# Autodesk Inventor assembly: USB_C_PD_PPS_sink_with_enclosure
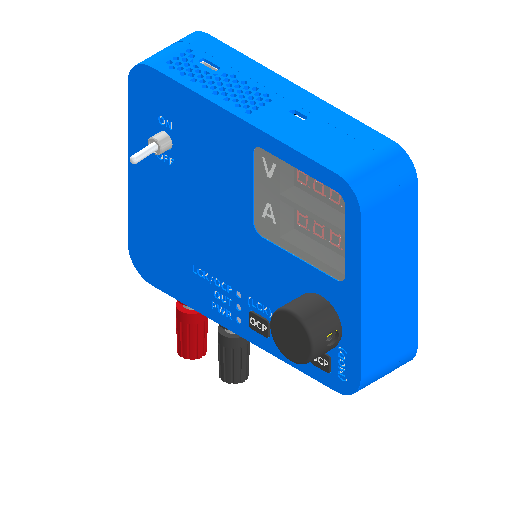
[picture p0: Inventor's stored thumbnail of the model, 512x512]
Saved by Autodesk Inventor 2025 (Build 290162000, 162)
## iProperties
Created: 2024-12-02
Part Number: USB_C_PD_PPS_sink_with_enclosure
Document SubType Name: Assembly
Designer: Jan Mareš
Author: Jan Mareš
## Documents named in this file (13)
- C:\Users\Jan Mareš\OneDrive - Vysoké učení technické v Brně\Dokumenty\Inventor\DP_PPS_USB_PD_enclosure\USB_C_PD_PPS_sink_with_enclosure.iam
- C:\Users\Jan Mareš\OneDrive - Vysoké učení technické v Brně\Dokumenty\Inventor\DP_PPS_USB_PD_enclosure\USB_C_PD_PPS_sink.iam
- C:\Users\Jan Mareš\OneDrive - Vysoké učení technické v Brně\Dokumenty\Inventor\DP_PPS_USB_PD_enclosure\top_enclosure.ipt
- C:\Users\Jan Mareš\OneDrive - Vysoké učení technické v Brně\Dokumenty\Inventor\DP_PPS_USB_PD_enclosure\STAUBLI_PK4-T_10017932.ipt
- C:\Users\Jan Mareš\OneDrive - Vysoké učení technické v Brně\Dokumenty\Inventor\DP_PPS_USB_PD_enclosure\Button cap.ipt
- C:\Users\Jan Mareš\OneDrive - Vysoké učení technické v Brně\Dokumenty\Inventor\DP_PPS_USB_PD_enclosure\Plexi-glass.ipt
- C:\Users\Jan Mareš\OneDrive - Vysoké učení technické v Brně\Dokumenty\Inventor\DP_PPS_USB_PD_enclosure\bottom_enclosure.ipt
- C:\Users\Jan Mareš\OneDrive - Vysoké učení technické v Brně\Dokumenty\Inventor\DP_PPS_USB_PD_enclosure\Aluminium_knob.ipt
- C:\Users\Jan Mareš\OneDrive - Vysoké učení technické v Brně\Dokumenty\Inventor\DP_PPS_USB_PD_enclosure\display_cover_2.ipt
- C:\Users\Jan Mareš\OneDrive - Vysoké učení technické v Brně\Dokumenty\Inventor\DP_PPS_USB_PD_enclosure\A_letter.ipt
- C:\Users\Jan Mareš\OneDrive - Vysoké učení technické v Brně\Dokumenty\Inventor\DP_PPS_USB_PD_enclosure\V_letter.ipt
- C:\Users\Jan Mareš\OneDrive - Vysoké učení technické v Brně\Dokumenty\Inventor\DP_PPS_USB_PD_enclosure\tilt_leg.ipt
- C:\Users\Jan Mareš\OneDrive - Vysoké učení technické v Brně\Dokumenty\Inventor\DP_PPS_USB_PD_enclosure\STAUBLI_PK4-T_10017932_red.ipt
## Components (16 placed, 12 different names)
1. USB_C_PD_PPS_sink:1 [sub-assembly] — Mate:1, Angle:1, Mate:2, Angle:2, Mate:3, Mate:9, Angle:3, Mate:10, Angle:4, Flush:1, Flush:2, Mate:11, Mate:24, Flush:5
2. top_enclosure:1 — Mate:3, Mate:7, Mate:23, Flush:4, Mate:25, Flush:6, Flush:7, Mate:26, Mate:27, Mate:28, Flush:8, Mate:29, Mate:30, Mate:31, Mate:33, Mate:34, Mate:36, Mate:37, Flush:9
3. bottom_enclosure:1 — Mate:23, Flush:4, Mate:38, Cylindrical:1, Mate:41, Mate:42, Mate:43, Flush:9
4. STAUBLI_PK4-T_10017932:2 — Mate:7, Mate:41
5. STAUBLI_PK4-T_10017932_red:1 — Mate:42, Mate:43
6. Aluminium_knob:1 — Mate:24, Flush:5, Mate:25
7. bottom_enclosure:2 — Flush:6, Flush:7, Mate:26
8. Plexi-glass:2 — Mate:27, Mate:28, Flush:8
9. display_cover_2:1 — Mate:29, Mate:30, Mate:31, Mate:32, Mate:35
10. A_letter:1 — Mate:32, Mate:33, Mate:34
11. V_letter:1 — Mate:35, Mate:36, Mate:37
12. Button cap:1 — Flush:1, Flush:2, Mate:11
13. Button cap:2
14. Button cap:3
15. tilt_leg:1 — Mate:38, Cylindrical:1
16. tilt_leg:2
## Component patterns: Buttons (3 elements), Tilt_legs (2 elements)
## Relationships (39: Mate 26, Flush 8, Angle 4, CylindricalJoint 1)
- Mate:1: USB_C_PD_PPS_sink:1
- Angle:1 (0 deg): USB_C_PD_PPS_sink:1
- Mate:2: USB_C_PD_PPS_sink:1
- Angle:2 (0 deg): USB_C_PD_PPS_sink:1
- Mate:3 (0.25 mm): USB_C_PD_PPS_sink:1 ↔ top_enclosure:1
- Mate:7: top_enclosure:1 ↔ STAUBLI_PK4-T_10017932:2
- Mate:9: USB_C_PD_PPS_sink:1
- Angle:3 (0 deg): USB_C_PD_PPS_sink:1
- Mate:10: USB_C_PD_PPS_sink:1
- Angle:4 (0 deg): USB_C_PD_PPS_sink:1
- Flush:1: USB_C_PD_PPS_sink:1 ↔ Button cap:1
- Flush:2: USB_C_PD_PPS_sink:1 ↔ Button cap:1
- Mate:11: USB_C_PD_PPS_sink:1 ↔ Button cap:1
- Mate:23: top_enclosure:1 ↔ bottom_enclosure:1
- Flush:4: top_enclosure:1 ↔ bottom_enclosure:1
- Mate:24: USB_C_PD_PPS_sink:1 ↔ Aluminium_knob:1
- Flush:5: USB_C_PD_PPS_sink:1 ↔ Aluminium_knob:1
- Mate:25 (0.4 mm): top_enclosure:1 ↔ Aluminium_knob:1
- Flush:6: top_enclosure:1 ↔ bottom_enclosure:2
- Flush:7: top_enclosure:1 ↔ bottom_enclosure:2
- Mate:26 (10 mm): top_enclosure:1 ↔ bottom_enclosure:2
- Mate:27: top_enclosure:1 ↔ Plexi-glass:2
- Mate:28: top_enclosure:1 ↔ Plexi-glass:2
- Flush:8: top_enclosure:1 ↔ Plexi-glass:2
- Mate:29 (0.1 mm): top_enclosure:1 ↔ display_cover_2:1
- Mate:30: top_enclosure:1 ↔ display_cover_2:1
- Mate:31: top_enclosure:1 ↔ display_cover_2:1
- Mate:32: display_cover_2:1 ↔ A_letter:1
- Mate:33: top_enclosure:1 ↔ A_letter:1
- Mate:34: top_enclosure:1 ↔ A_letter:1
- Mate:35: display_cover_2:1 ↔ V_letter:1
- Mate:36: top_enclosure:1 ↔ V_letter:1
- Mate:37: top_enclosure:1 ↔ V_letter:1
- Mate:38: bottom_enclosure:1 ↔ tilt_leg:1
- Cylindrical:1: bottom_enclosure:1 ↔ tilt_leg:1
- Mate:41: bottom_enclosure:1 ↔ STAUBLI_PK4-T_10017932:2
- Mate:42: bottom_enclosure:1 ↔ STAUBLI_PK4-T_10017932_red:1
- Mate:43: bottom_enclosure:1 ↔ STAUBLI_PK4-T_10017932_red:1
- Flush:9: top_enclosure:1 ↔ bottom_enclosure:1
## Named parameters: offset_top_e = 0.25 mm
